# Autodesk Inventor assembly: Four cylinder Engine Assembly
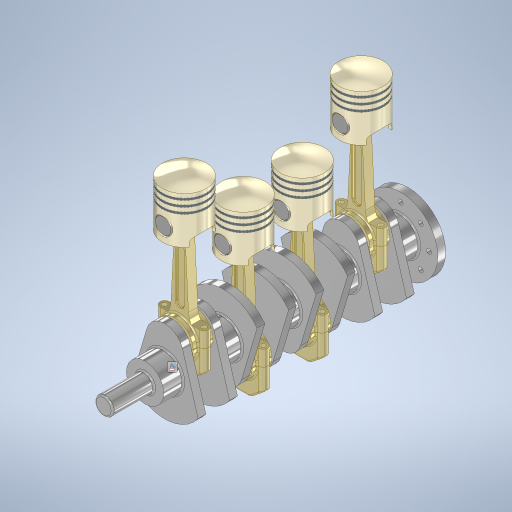
[picture p0: Inventor's stored thumbnail of the model, 512x512]
Saved by Autodesk Inventor 2023 (Build 270158000, 158)
## iProperties
Created: 2023-10-21
Part Number: Four cylinder Engine Assembly
Document SubType Name: Assembly
Designer: Beatrice
Author: Beatrice
## Documents named in this file (5)
- C:\Users\Beatrice\Documents\Inventor\4_Cylinder_Engine\4 cylinder engine assembly\Four cylinder Engine Assembly.iam
- C:\Users\Beatrice\Documents\Inventor\4_Cylinder_Engine\4 cylinder engine assembly\Base sketch of Main_Assembly.ipt
- C:\Users\Beatrice\Documents\Inventor\4_Cylinder_Engine\4 cylinder engine assembly\crankshaft.ipt
- C:\Users\Beatrice\Documents\Inventor\4_Cylinder_Engine\4 cylinder engine assembly\connecting_rod_sub_Assembly.iam
- C:\Users\Beatrice\Documents\Inventor\4_Cylinder_Engine\4 cylinder engine assembly\piston_sub_assembly.iam
## Components (10 placed, 4 different names)
1. Base sketch of Main_Assembly:1 — Mate:1, Flush:1, Mate:2, Mate:3, Drive_, Mate:7, Mate:8, Mate:12, Mate:13, Mate:14, Mate:15
2. crankshaft:1 — Mate:1, Flush:1, Mate:5, Drive_, Mate:9, Mate:16, Mate:17
3. connecting_rod_sub_Assembly:1 [sub-assembly] — Mate:4, Insert:1, Mate:5
4. piston_sub_assembly:1 [sub-assembly] — Mate:2, Mate:3, Mate:4, Insert:1
5. connecting_rod_sub_Assembly:2 [sub-assembly] — Mate:6, Insert:2, Mate:9
6. piston_sub_assembly:2 [sub-assembly] — Mate:6, Insert:2, Mate:7, Mate:8
7. connecting_rod_sub_Assembly:3 [sub-assembly] — Mate:10, Insert:3, Mate:16
8. piston_sub_assembly:3 [sub-assembly] — Mate:10, Insert:3, Mate:12, Mate:14
9. connecting_rod_sub_Assembly:4 [sub-assembly] — Mate:11, Insert:4, Mate:17
10. piston_sub_assembly:4 [sub-assembly] — Mate:11, Insert:4, Mate:13, Mate:15
## Relationships (23: Mate 17, Insert 4, Flush 1, Angle 1)
- Mate:1: Base sketch of Main_Assembly:1 ↔ crankshaft:1
- Flush:1: Base sketch of Main_Assembly:1 ↔ crankshaft:1
- Mate:2: Base sketch of Main_Assembly:1 ↔ piston_sub_assembly:1
- Mate:3: Base sketch of Main_Assembly:1 ↔ piston_sub_assembly:1
- Mate:4: connecting_rod_sub_Assembly:1 ↔ piston_sub_assembly:1
- Insert:1: connecting_rod_sub_Assembly:1 ↔ piston_sub_assembly:1
- Mate:5: crankshaft:1 ↔ connecting_rod_sub_Assembly:1
- Drive_ [Angle] (180 deg): Base sketch of Main_Assembly:1 ↔ crankshaft:1
- Mate:6: connecting_rod_sub_Assembly:2 ↔ piston_sub_assembly:2
- Insert:2: connecting_rod_sub_Assembly:2 ↔ piston_sub_assembly:2
- Mate:7: Base sketch of Main_Assembly:1 ↔ piston_sub_assembly:2
- Mate:8: Base sketch of Main_Assembly:1 ↔ piston_sub_assembly:2
- Mate:9: crankshaft:1 ↔ connecting_rod_sub_Assembly:2
- Mate:10: connecting_rod_sub_Assembly:3 ↔ piston_sub_assembly:3
- Mate:11: connecting_rod_sub_Assembly:4 ↔ piston_sub_assembly:4
- Insert:3: connecting_rod_sub_Assembly:3 ↔ piston_sub_assembly:3
- Insert:4: connecting_rod_sub_Assembly:4 ↔ piston_sub_assembly:4
- Mate:12: Base sketch of Main_Assembly:1 ↔ piston_sub_assembly:3
- Mate:13: Base sketch of Main_Assembly:1 ↔ piston_sub_assembly:4
- Mate:14: Base sketch of Main_Assembly:1 ↔ piston_sub_assembly:3
- Mate:15: Base sketch of Main_Assembly:1 ↔ piston_sub_assembly:4
- Mate:16: crankshaft:1 ↔ connecting_rod_sub_Assembly:3
- Mate:17: crankshaft:1 ↔ connecting_rod_sub_Assembly:4
